# Autodesk Inventor assembly: Wall Assembly 1600 - 175 - 23 pieces
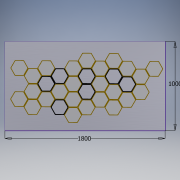
[picture p0: Inventor's stored thumbnail of the model, 180x180]
Saved by Autodesk Inventor 2019 (Build 230136000, 136)
## iProperties
Created: 2021-07-14
Part Number: Wall Assembly 1600 - 175 - 23 pieces
Document SubType Name: Assembly
Designer: Lix
Author: Lix
## Documents named in this file (4)
- G:\Project\Hybrids\HexaWall\Inventor\Wall Assembly 1600 - 175 - 23 pieces - version B.iam
- G:\Project\Hybrids\HexaWall\Inventor\Wall - 160x70.ipt
- G:\Project\Hybrids\HexaWall\Inventor\Hexagonal Deco Lamp Assembly 175.iam
- G:\Project\Hybrids\HexaWall\Inventor\Flat Placeholder v1 - 175 - 8mm rim.ipt
## Components (34 placed, 3 different names)
1. Wall - 160x70:1 — Mate:2, Mate:39, Mate:40, Mate:43, Mate:46, Mate:49, Mate:50, Mate:55, Mate:84, Mate:87, Mate:90, Mate:93, Mate:96
2. Hexagonal Deco Lamp Assembly 175:1 [sub-assembly] — Flush:1, Flush:2, Flush:3, Flush:4, Mate:4, Mate:14, Mate:62, Mate:64, Mate:85
3. Hexagonal Deco Lamp Assembly 175:2 [sub-assembly] — Flush:1, Mate:2, Mate:6, Mate:8, Mate:10, Mate:42, Mate:59, Mate:60, Mate:62
4. Hexagonal Deco Lamp Assembly 175:3 [sub-assembly] — Flush:2, Mate:4, Mate:6, Mate:61
5. Hexagonal Deco Lamp Assembly 175:4 [sub-assembly] — Flush:3, Flush:6, Mate:12, Mate:57, Mate:58
6. Hexagonal Deco Lamp Assembly 175:5 [sub-assembly] — Flush:5, Mate:10, Mate:12, Mate:41, Mate:58, Mate:59, Mate:76, Mate:77
7. Hexagonal Deco Lamp Assembly 175:6 [sub-assembly] — Flush:4, Flush:5, Mate:8, Mate:60, Mate:61
8. Hexagonal Deco Lamp Assembly 175:7 [sub-assembly] — Flush:6, Flush:7, Flush:9, Mate:14, Mate:16, Mate:18, Mate:45, Mate:63, Mate:64, Mate:65, Mate:82, Mate:83
9. Hexagonal Deco Lamp Assembly 175:8 [sub-assembly] — Flush:7, Flush:8, Flush:9, Mate:16, Mate:63, Mate:91
10. Hexagonal Deco Lamp Assembly 175:9 [sub-assembly] — Flush:8, Flush:10, Mate:18, Mate:20, Mate:65, Mate:66, Mate:86, Mate:89
11. Hexagonal Deco Lamp Assembly 175:10 [sub-assembly] — Flush:11, Flush:12, Mate:22, Mate:24, Mate:26, Mate:28, Mate:67, Mate:68, Mate:69
12. Hexagonal Deco Lamp Assembly 175:11 [sub-assembly] — Flush:13, Flush:14, Flush:15, Mate:24, Mate:30, Mate:51, Mate:69, Mate:70, Mate:71
13. Hexagonal Deco Lamp Assembly 175:12 [sub-assembly] — Flush:15, Flush:16, Mate:30, Mate:32, Mate:47, Mate:70, Mate:72
14. Hexagonal Deco Lamp Assembly 175:13 [sub-assembly] — Flush:14, Mate:28, Mate:68
15. Hexagonal Deco Lamp Assembly 175:14 [sub-assembly] — Flush:10, Flush:11, Mate:20, Mate:22, Mate:53, Mate:66, Mate:67, Mate:88
16. Hexagonal Deco Lamp Assembly 175:15 [sub-assembly] — Flush:12, Flush:13, Mate:26, Mate:54, Mate:71, Mate:78, Mate:79, Mate:98
17. Hexagonal Deco Lamp Assembly 175:16 [sub-assembly] — Flush:16, Flush:17, Flush:18, Mate:32, Mate:34, Mate:72, Mate:73
18. Hexagonal Deco Lamp Assembly 175:17 [sub-assembly] — Flush:17, Flush:18, Flush:19, Mate:34, Mate:36, Mate:38, Mate:48, Mate:73, Mate:74, Mate:75
19. Hexagonal Deco Lamp Assembly 175:18 [sub-assembly] — Flush:19, Mate:36, Mate:52, Mate:75
20. Hexagonal Deco Lamp Assembly 175:19 [sub-assembly] — Mate:38, Mate:39, Mate:74
21. Flat Placeholder v1 - 175 - 8mm rim:1 — Mate:40, Mate:41, Mate:42, Mate:44
22. Flat Placeholder v1 - 175 - 8mm rim:2 — Mate:43, Mate:44, Mate:45, Mate:56, Mate:92
23. Flat Placeholder v1 - 175 - 8mm rim:3 — Mate:46, Mate:47, Mate:48
24. Flat Placeholder v1 - 175 - 8mm rim:4 — Mate:50, Mate:53, Mate:54
25. Flat Placeholder v1 - 175 - 8mm rim:5 — Mate:49, Mate:51, Mate:52
26. Flat Placeholder v1 - 175 - 8mm rim:6 — Mate:55, Mate:56, Mate:57
27. Hexagonal Deco Lamp Assembly 175:20 [sub-assembly] — Mate:76, Mate:77
28. Hexagonal Deco Lamp Assembly 175:21 [sub-assembly] — Mate:78, Mate:79, Mate:80, Mate:81, Mate:95
29. Hexagonal Deco Lamp Assembly 175:22 [sub-assembly] — Mate:80, Mate:81
30. Hexagonal Deco Lamp Assembly 175:23 [sub-assembly] — Mate:82, Mate:83, Mate:84, Mate:88, Mate:89
31. Flat Placeholder v1 - 175 - 8mm rim:7 — Mate:85, Mate:86, Mate:87
32. Hexagonal Deco Lamp Assembly 175:24 [sub-assembly] — Mate:90, Mate:91, Mate:92, Mate:94
33. Hexagonal Deco Lamp Assembly 175:25 [sub-assembly] — Mate:93, Mate:94, Mate:95, Mate:97
34. Flat Placeholder v1 - 175 - 8mm rim:8 — Mate:96, Mate:97, Mate:98
## Relationships (98: Mate 79, Flush 19)
- Flush:1: Hexagonal Deco Lamp Assembly 175:1 ↔ Hexagonal Deco Lamp Assembly 175:2
- Flush:2: Hexagonal Deco Lamp Assembly 175:1 ↔ Hexagonal Deco Lamp Assembly 175:3
- Flush:3: Hexagonal Deco Lamp Assembly 175:1 ↔ Hexagonal Deco Lamp Assembly 175:4
- Flush:4: Hexagonal Deco Lamp Assembly 175:1 ↔ Hexagonal Deco Lamp Assembly 175:6
- Flush:5: Hexagonal Deco Lamp Assembly 175:5 ↔ Hexagonal Deco Lamp Assembly 175:6
- Flush:6: Hexagonal Deco Lamp Assembly 175:4 ↔ Hexagonal Deco Lamp Assembly 175:7
- Flush:7: Hexagonal Deco Lamp Assembly 175:7 ↔ Hexagonal Deco Lamp Assembly 175:8
- Flush:8: Hexagonal Deco Lamp Assembly 175:8 ↔ Hexagonal Deco Lamp Assembly 175:9
- Flush:9: Hexagonal Deco Lamp Assembly 175:7 ↔ Hexagonal Deco Lamp Assembly 175:8
- Flush:10: Hexagonal Deco Lamp Assembly 175:9 ↔ Hexagonal Deco Lamp Assembly 175:14
- Flush:11: Hexagonal Deco Lamp Assembly 175:10 ↔ Hexagonal Deco Lamp Assembly 175:14
- Flush:12: Hexagonal Deco Lamp Assembly 175:10 ↔ Hexagonal Deco Lamp Assembly 175:15
- Flush:13: Hexagonal Deco Lamp Assembly 175:11 ↔ Hexagonal Deco Lamp Assembly 175:15
- Flush:14: Hexagonal Deco Lamp Assembly 175:11 ↔ Hexagonal Deco Lamp Assembly 175:13
- Flush:15: Hexagonal Deco Lamp Assembly 175:11 ↔ Hexagonal Deco Lamp Assembly 175:12
- Flush:16: Hexagonal Deco Lamp Assembly 175:12 ↔ Hexagonal Deco Lamp Assembly 175:16
- Flush:17: Hexagonal Deco Lamp Assembly 175:16 ↔ Hexagonal Deco Lamp Assembly 175:17
- Flush:18: Hexagonal Deco Lamp Assembly 175:16 ↔ Hexagonal Deco Lamp Assembly 175:17
- Flush:19: Hexagonal Deco Lamp Assembly 175:17 ↔ Hexagonal Deco Lamp Assembly 175:18
- Mate:2: Wall - 160x70:1 ↔ Hexagonal Deco Lamp Assembly 175:2
- Mate:4: Hexagonal Deco Lamp Assembly 175:1 ↔ Hexagonal Deco Lamp Assembly 175:3
- Mate:6: Hexagonal Deco Lamp Assembly 175:2 ↔ Hexagonal Deco Lamp Assembly 175:3
- Mate:8: Hexagonal Deco Lamp Assembly 175:2 ↔ Hexagonal Deco Lamp Assembly 175:6
- Mate:10: Hexagonal Deco Lamp Assembly 175:2 ↔ Hexagonal Deco Lamp Assembly 175:5
- Mate:12: Hexagonal Deco Lamp Assembly 175:4 ↔ Hexagonal Deco Lamp Assembly 175:5
- Mate:14: Hexagonal Deco Lamp Assembly 175:1 ↔ Hexagonal Deco Lamp Assembly 175:7
- Mate:16: Hexagonal Deco Lamp Assembly 175:7 ↔ Hexagonal Deco Lamp Assembly 175:8
- Mate:18: Hexagonal Deco Lamp Assembly 175:7 ↔ Hexagonal Deco Lamp Assembly 175:9
- Mate:20: Hexagonal Deco Lamp Assembly 175:9 ↔ Hexagonal Deco Lamp Assembly 175:14
- Mate:22: Hexagonal Deco Lamp Assembly 175:10 ↔ Hexagonal Deco Lamp Assembly 175:14
- Mate:24: Hexagonal Deco Lamp Assembly 175:10 ↔ Hexagonal Deco Lamp Assembly 175:11
- Mate:26: Hexagonal Deco Lamp Assembly 175:10 ↔ Hexagonal Deco Lamp Assembly 175:15
- Mate:28: Hexagonal Deco Lamp Assembly 175:10 ↔ Hexagonal Deco Lamp Assembly 175:13
- Mate:30: Hexagonal Deco Lamp Assembly 175:11 ↔ Hexagonal Deco Lamp Assembly 175:12
- Mate:32: Hexagonal Deco Lamp Assembly 175:12 ↔ Hexagonal Deco Lamp Assembly 175:16
- Mate:34: Hexagonal Deco Lamp Assembly 175:16 ↔ Hexagonal Deco Lamp Assembly 175:17
- Mate:36: Hexagonal Deco Lamp Assembly 175:17 ↔ Hexagonal Deco Lamp Assembly 175:18
- Mate:38: Hexagonal Deco Lamp Assembly 175:17 ↔ Hexagonal Deco Lamp Assembly 175:19
- Mate:39: Wall - 160x70:1 ↔ Hexagonal Deco Lamp Assembly 175:19
- Mate:40: Wall - 160x70:1 ↔ Flat Placeholder v1 - 175 - 8mm rim:1
- Mate:41: Hexagonal Deco Lamp Assembly 175:5 ↔ Flat Placeholder v1 - 175 - 8mm rim:1
- Mate:42: Hexagonal Deco Lamp Assembly 175:2 ↔ Flat Placeholder v1 - 175 - 8mm rim:1
- Mate:43: Wall - 160x70:1 ↔ Flat Placeholder v1 - 175 - 8mm rim:2
- Mate:44: Flat Placeholder v1 - 175 - 8mm rim:1 ↔ Flat Placeholder v1 - 175 - 8mm rim:2
- Mate:45: Hexagonal Deco Lamp Assembly 175:7 ↔ Flat Placeholder v1 - 175 - 8mm rim:2
- Mate:46: Wall - 160x70:1 ↔ Flat Placeholder v1 - 175 - 8mm rim:3
- Mate:47: Hexagonal Deco Lamp Assembly 175:12 ↔ Flat Placeholder v1 - 175 - 8mm rim:3
- Mate:48: Hexagonal Deco Lamp Assembly 175:17 ↔ Flat Placeholder v1 - 175 - 8mm rim:3
- Mate:49: Wall - 160x70:1 ↔ Flat Placeholder v1 - 175 - 8mm rim:5
- Mate:50: Wall - 160x70:1 ↔ Flat Placeholder v1 - 175 - 8mm rim:4
- Mate:51: Hexagonal Deco Lamp Assembly 175:11 ↔ Flat Placeholder v1 - 175 - 8mm rim:5
- Mate:52: Hexagonal Deco Lamp Assembly 175:18 ↔ Flat Placeholder v1 - 175 - 8mm rim:5
- Mate:53: Hexagonal Deco Lamp Assembly 175:14 ↔ Flat Placeholder v1 - 175 - 8mm rim:4
- Mate:54: Hexagonal Deco Lamp Assembly 175:15 ↔ Flat Placeholder v1 - 175 - 8mm rim:4
- Mate:55: Wall - 160x70:1 ↔ Flat Placeholder v1 - 175 - 8mm rim:6
- Mate:56: Flat Placeholder v1 - 175 - 8mm rim:2 ↔ Flat Placeholder v1 - 175 - 8mm rim:6
- Mate:57: Hexagonal Deco Lamp Assembly 175:4 ↔ Flat Placeholder v1 - 175 - 8mm rim:6
- Mate:58: Hexagonal Deco Lamp Assembly 175:4 ↔ Hexagonal Deco Lamp Assembly 175:5
- Mate:59: Hexagonal Deco Lamp Assembly 175:2 ↔ Hexagonal Deco Lamp Assembly 175:5
- Mate:60: Hexagonal Deco Lamp Assembly 175:2 ↔ Hexagonal Deco Lamp Assembly 175:6
- Mate:61: Hexagonal Deco Lamp Assembly 175:3 ↔ Hexagonal Deco Lamp Assembly 175:6
- Mate:62: Hexagonal Deco Lamp Assembly 175:1 ↔ Hexagonal Deco Lamp Assembly 175:2
- Mate:63: Hexagonal Deco Lamp Assembly 175:7 ↔ Hexagonal Deco Lamp Assembly 175:8
- Mate:64: Hexagonal Deco Lamp Assembly 175:1 ↔ Hexagonal Deco Lamp Assembly 175:7
- Mate:65: Hexagonal Deco Lamp Assembly 175:7 ↔ Hexagonal Deco Lamp Assembly 175:9
- Mate:66: Hexagonal Deco Lamp Assembly 175:9 ↔ Hexagonal Deco Lamp Assembly 175:14
- Mate:67: Hexagonal Deco Lamp Assembly 175:10 ↔ Hexagonal Deco Lamp Assembly 175:14
- Mate:68: Hexagonal Deco Lamp Assembly 175:10 ↔ Hexagonal Deco Lamp Assembly 175:13
- Mate:69: Hexagonal Deco Lamp Assembly 175:10 ↔ Hexagonal Deco Lamp Assembly 175:11
- Mate:70: Hexagonal Deco Lamp Assembly 175:11 ↔ Hexagonal Deco Lamp Assembly 175:12
- Mate:71: Hexagonal Deco Lamp Assembly 175:11 ↔ Hexagonal Deco Lamp Assembly 175:15
- Mate:72: Hexagonal Deco Lamp Assembly 175:12 ↔ Hexagonal Deco Lamp Assembly 175:16
- Mate:73: Hexagonal Deco Lamp Assembly 175:16 ↔ Hexagonal Deco Lamp Assembly 175:17
- Mate:74: Hexagonal Deco Lamp Assembly 175:17 ↔ Hexagonal Deco Lamp Assembly 175:19
- Mate:75: Hexagonal Deco Lamp Assembly 175:17 ↔ Hexagonal Deco Lamp Assembly 175:18
- Mate:76: Hexagonal Deco Lamp Assembly 175:5 ↔ Hexagonal Deco Lamp Assembly 175:20
- Mate:77: Hexagonal Deco Lamp Assembly 175:5 ↔ Hexagonal Deco Lamp Assembly 175:20
- Mate:78: Hexagonal Deco Lamp Assembly 175:15 ↔ Hexagonal Deco Lamp Assembly 175:21
- Mate:79: Hexagonal Deco Lamp Assembly 175:15 ↔ Hexagonal Deco Lamp Assembly 175:21
- Mate:80: Hexagonal Deco Lamp Assembly 175:21 ↔ Hexagonal Deco Lamp Assembly 175:22
- Mate:81: Hexagonal Deco Lamp Assembly 175:21 ↔ Hexagonal Deco Lamp Assembly 175:22
- Mate:82: Hexagonal Deco Lamp Assembly 175:7 ↔ Hexagonal Deco Lamp Assembly 175:23
- Mate:83: Hexagonal Deco Lamp Assembly 175:7 ↔ Hexagonal Deco Lamp Assembly 175:23
- Mate:84: Wall - 160x70:1 ↔ Hexagonal Deco Lamp Assembly 175:23
- Mate:85: Hexagonal Deco Lamp Assembly 175:1 ↔ Flat Placeholder v1 - 175 - 8mm rim:7
- Mate:86: Hexagonal Deco Lamp Assembly 175:9 ↔ Flat Placeholder v1 - 175 - 8mm rim:7
- Mate:87: Wall - 160x70:1 ↔ Flat Placeholder v1 - 175 - 8mm rim:7
- Mate:88: Hexagonal Deco Lamp Assembly 175:14 ↔ Hexagonal Deco Lamp Assembly 175:23
- Mate:89: Hexagonal Deco Lamp Assembly 175:9 ↔ Hexagonal Deco Lamp Assembly 175:23
- Mate:90: Wall - 160x70:1 ↔ Hexagonal Deco Lamp Assembly 175:24
- Mate:91: Hexagonal Deco Lamp Assembly 175:8 ↔ Hexagonal Deco Lamp Assembly 175:24
- Mate:92: Flat Placeholder v1 - 175 - 8mm rim:2 ↔ Hexagonal Deco Lamp Assembly 175:24
- Mate:93: Wall - 160x70:1 ↔ Hexagonal Deco Lamp Assembly 175:25
- Mate:94: Hexagonal Deco Lamp Assembly 175:24 ↔ Hexagonal Deco Lamp Assembly 175:25
- Mate:95: Hexagonal Deco Lamp Assembly 175:21 ↔ Hexagonal Deco Lamp Assembly 175:25
- Mate:96: Wall - 160x70:1 ↔ Flat Placeholder v1 - 175 - 8mm rim:8
- Mate:97: Hexagonal Deco Lamp Assembly 175:25 ↔ Flat Placeholder v1 - 175 - 8mm rim:8
- Mate:98: Hexagonal Deco Lamp Assembly 175:15 ↔ Flat Placeholder v1 - 175 - 8mm rim:8
